# Autodesk Inventor assembly: DržačiSaSenzorimaUdaljenosti_v.1.0
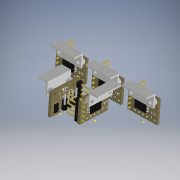
[picture p0: Inventor's stored thumbnail of the model, 180x180]
Saved by Autodesk Inventor 2020 (Build 240168000, 168)
## iProperties
Created: 2020-07-11
Part Number: DržačiSaSenzorimaUdaljenosti_v.1.0
Document SubType Name: Assembly
Designer: Sičaja
Author: Sičaja
## Documents named in this file (3)
- C:\Users\Sicaja\Documents\Draws_Inventor\Robocup_robot\DržačiSaSenzorimaUdaljenosti_v.1.0.iam
- C:\Users\Sicaja\Documents\Draws_Inventor\Robocup_robot\DržačSenzoraUdaljenostiOnlyOne(1)_v.1.0.ipt
- C:\Users\Sicaja\Documents\Draws_Inventor\Robocup_robot\mrm-lid-an.ipt
## Components (10 placed, 2 different names)
1. DržačSenzoraUdaljenostiOnlyOne(1)_v.1.0:2 — Mate:2, Mate:3, Insert:7, Insert:8
2. DržačSenzoraUdaljenostiOnlyOne(1)_v.1.0:3 — Mate:4, Mate:5, Insert:9, Insert:10
3. mrm-lid-an:1 — Insert:7, Insert:8
4. mrm-lid-an:2 — Insert:9, Insert:10
5. mrm-lid-an:3 — Insert:3, Insert:4
6. mrm-lid-an:4 — Insert:5, Insert:6
7. mrm-lid-an:5 — Insert:1, Insert:2
8. DržačSenzoraUdaljenostiOnlyOne(1)_v.1.0:1 — Mate:4, Mate:5, Insert:1, Insert:2
9. DržačSenzoraUdaljenostiOnlyOne(1)_v.1.0:4 — Insert:3, Insert:4
10. DržačSenzoraUdaljenostiOnlyOne(1)_v.1.0:5 — Mate:2, Mate:3, Insert:5, Insert:6
## Component patterns: (3 elements, first: DržačSenzoraUdaljenostiOnlyOne(1)_v.1.0:1)
## Relationships (14: Insert 10, Mate 4)
- Mate:2: DržačSenzoraUdaljenostiOnlyOne(1)_v.1.0:2 ↔ DržačSenzoraUdaljenostiOnlyOne(1)_v.1.0:5
- Mate:3: DržačSenzoraUdaljenostiOnlyOne(1)_v.1.0:2 ↔ DržačSenzoraUdaljenostiOnlyOne(1)_v.1.0:5
- Mate:4: DržačSenzoraUdaljenostiOnlyOne(1)_v.1.0:3 ↔ DržačSenzoraUdaljenostiOnlyOne(1)_v.1.0:1
- Mate:5: DržačSenzoraUdaljenostiOnlyOne(1)_v.1.0:3 ↔ DržačSenzoraUdaljenostiOnlyOne(1)_v.1.0:1
- Insert:1: mrm-lid-an:5 ↔ DržačSenzoraUdaljenostiOnlyOne(1)_v.1.0:1
- Insert:2: mrm-lid-an:5 ↔ DržačSenzoraUdaljenostiOnlyOne(1)_v.1.0:1
- Insert:3: mrm-lid-an:3 ↔ DržačSenzoraUdaljenostiOnlyOne(1)_v.1.0:4
- Insert:4: mrm-lid-an:3 ↔ DržačSenzoraUdaljenostiOnlyOne(1)_v.1.0:4
- Insert:5: mrm-lid-an:4 ↔ DržačSenzoraUdaljenostiOnlyOne(1)_v.1.0:5
- Insert:6: mrm-lid-an:4 ↔ DržačSenzoraUdaljenostiOnlyOne(1)_v.1.0:5
- Insert:7: DržačSenzoraUdaljenostiOnlyOne(1)_v.1.0:2 ↔ mrm-lid-an:1
- Insert:8: DržačSenzoraUdaljenostiOnlyOne(1)_v.1.0:2 ↔ mrm-lid-an:1
- Insert:9: DržačSenzoraUdaljenostiOnlyOne(1)_v.1.0:3 ↔ mrm-lid-an:2
- Insert:10: DržačSenzoraUdaljenostiOnlyOne(1)_v.1.0:3 ↔ mrm-lid-an:2
